# Autodesk Inventor assembly: FrostyCarbonCoin25t-V6-SurfaceAreaModel
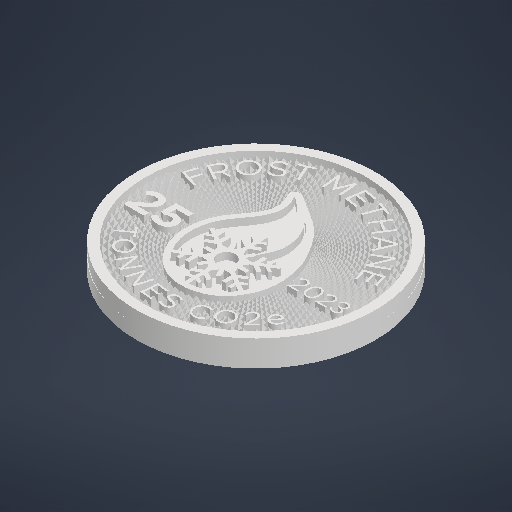
[picture p0: Inventor's stored thumbnail of the model, 512x512]
Saved by Autodesk Inventor 2026.1 (Build 301233020, 233B)
## iProperties
Created: 2026-01-26
Part Number: FrostyCarbonCoin25t-V6-SurfaceAreaModel
Document SubType Name: Assembly
Designer: incep
Mass: 7.82603 g
Surface Area: 119.444 cm^2
Volume: 7.82603 cm^3
Density: 1 g/cm^3
Author: incep
## Documents named in this file (3)
- C:\Projects\FrostyCarbonCoin\FrostyCarbonCoin25t-V6-SurfaceAreaModel.iam
- C:\Projects\FrostyCarbonCoin\FrostyCarbonCoin25t-V6-Front-SurfaceAreaModel.ipt
- C:\Projects\FrostyCarbonCoin\FrostyCarbonCoin25t-V6-Back-SurfaceAreaModel.ipt
## Components (2 placed, 2 different names)
1. FrostyCarbonCoin25t-V6-Front-SurfaceAreaModel:1 — Flush:1, Flush:2, Flush:3, Mate:1, Mate:2, Mate:3, Mate:4, Mate:5, Mate:7
2. FrostyCarbonCoin25t-V6-Back-SurfaceAreaModel:1 — Flush:4, Flush:5, Mate:6, Mate:7
## Relationships (12: Mate 7, Flush 5)
- Flush:1: FrostyCarbonCoin25t-V6-Front-SurfaceAreaModel:1
- Flush:2: FrostyCarbonCoin25t-V6-Front-SurfaceAreaModel:1
- Flush:3: FrostyCarbonCoin25t-V6-Front-SurfaceAreaModel:1
- Mate:1: FrostyCarbonCoin25t-V6-Front-SurfaceAreaModel:1
- Mate:2: FrostyCarbonCoin25t-V6-Front-SurfaceAreaModel:1
- Mate:3: FrostyCarbonCoin25t-V6-Front-SurfaceAreaModel:1
- Mate:4: FrostyCarbonCoin25t-V6-Front-SurfaceAreaModel:1
- Mate:5: FrostyCarbonCoin25t-V6-Front-SurfaceAreaModel:1
- Flush:4: FrostyCarbonCoin25t-V6-Back-SurfaceAreaModel:1
- Flush:5: FrostyCarbonCoin25t-V6-Back-SurfaceAreaModel:1
- Mate:6: FrostyCarbonCoin25t-V6-Back-SurfaceAreaModel:1
- Mate:7: FrostyCarbonCoin25t-V6-Front-SurfaceAreaModel:1 ↔ FrostyCarbonCoin25t-V6-Back-SurfaceAreaModel:1
